# Autodesk Inventor assembly: Right Angle Structure
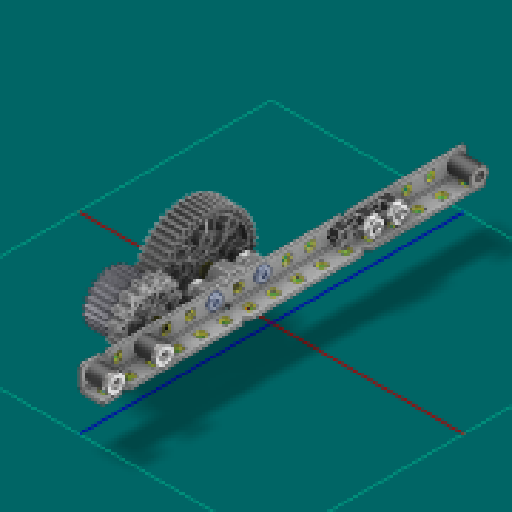
[picture p0: Inventor's stored thumbnail of the model, 512x512]
Saved by Autodesk Inventor 2025 (Build 290162000, 162)
## iProperties
Created: 2024-10-20
Part Number: Right Angle Structure
Document SubType Name: Assembly
Designer: Averey Ku
Author: Averey Ku
## Documents named in this file (18)
- C:\Users\avere\VEX\High Stakes\CAD\V2\Intake\Right Angle Structure\Right Angle Structure.iam
- C:\Users\avere\VEX\High Stakes\CAD\V2\Intake\Right Angle Structure\Right Alu Angle 1x1x16.ipt
- C:\Users\avere\VEX\High Stakes\CAD\V2\Intake\Right Angle Structure\Right Bearing Flat NScrew Slotted Offset.iam
- C:\Users\avere\VEX\High Stakes\CAD\ROBOPROS-CAD-Inventor\Motion\Spacers\Spacer Nylon .375 OD\NSpacer .375 OD x .500.ipt
- D:\VEX\High Stakes\CAD\ROBOPROS-CAD-Inventor\Motion\Spacers\Spacer Nylon .375 OD.ipt
- C:\Users\avere\VEX\High Stakes\CAD\ROBOPROS-CAD-Inventor\Motion\Spacers\Washer Steel\SWasher .375 OD x .015625.ipt
- D:\VEX\High Stakes\CAD\ROBOPROS-CAD-Inventor\Motion\Spacers\Washer Steel.ipt
- C:\Users\avere\VEX\High Stakes\CAD\V2\Intake\Right Angle Structure\Right HS Bearing Flat.ipt
- C:\Users\avere\VEX\High Stakes\CAD\ROBOPROS-CAD-Inventor\Structure\Hardware\Screw Shoulder Robosource\SScrew Shoulder Smooth .500 x .04.ipt
- D:\VEX\High Stakes\CAD\ROBOPROS-CAD-Inventor\Structure\Hardware\Screw Shoulder Robosource.ipt
- C:\Users\avere\VEX\High Stakes\CAD\ROBOPROS-CAD-Inventor\Structure\Hardware\Nut Nylon\Nut Nylon - White.ipt
- D:\VEX\High Stakes\CAD\ROBOPROS-CAD-Inventor\Structure\Hardware\Nut Nylon.ipt
- C:\Users\avere\VEX\High Stakes\CAD\ROBOPROS-CAD-Inventor\Motion\Spacers\Spacer Nylon .375 OD\NSpacer .375 OD x .375.ipt
- C:\Users\avere\VEX\High Stakes\CAD\ROBOPROS-CAD-Inventor\Motion\Spacers\Washer Steel\SWasher .375 OD x .062500.ipt
- C:\Users\avere\VEX\High Stakes\CAD\ROBOPROS-CAD-Inventor\Motion\Spacers\Washer Teflon\TWasher .375 OD x .04000.ipt
- D:\VEX\High Stakes\CAD\ROBOPROS-CAD-Inventor\Motion\Spacers\Washer Teflon.ipt
- C:\Users\avere\VEX\High Stakes\CAD\V2\Intake\Gearbox.iam
- Gearbox Left.iam
## Components (16 placed, 11 different names)
1. Right Alu Angle 1x1x16:1 — Mate:2, Mate:1, Flush:1, Mate:3, Insert:1, Insert:3, Mate:4, Insert:4, Insert:7, Insert:8, Insert:11, Insert:14, Insert:15
2. Right Bearing Flat NScrew Slotted Offset:1 [sub-assembly] — Mate:3, Insert:1
3. NSpacer .375 OD x .500:1 — Insert:3, Insert:2
4. SWasher .375 OD x .015625:1 — Insert:2
5. Right HS Bearing Flat:1 — Mate:4, Insert:4, Insert:5, Insert:6, Mate:6
6. SScrew Shoulder Smooth .500 x .04:1 — Insert:7
7. SScrew Shoulder Smooth .500 x .04:2 — Insert:8
8. Nut Nylon - White:1 — Insert:5
9. Nut Nylon - White:2 — Insert:6
10. NSpacer .375 OD x .375:2 — Insert:11, Insert:10
11. SWasher .375 OD x .062500:2 — Insert:10, Insert:9
12. TWasher .375 OD x .04000:1 — Insert:9
13. NSpacer .375 OD x .375:3 — Insert:14, Insert:13
14. SWasher .375 OD x .062500:3 — Insert:13, Insert:12
15. TWasher .375 OD x .04000:2 — Insert:12
16. Gearbox Left:1 [sub-assembly] — Insert:15, Mate:6
## Relationships (21: Insert 15, Mate 6)
- Mate:2: Right Alu Angle 1x1x16:1
- Mate:1: Right Alu Angle 1x1x16:1
- Flush:1 [Mate] (-101.6 mm): Right Alu Angle 1x1x16:1
- Mate:3: Right Alu Angle 1x1x16:1 ↔ Right Bearing Flat NScrew Slotted Offset:1
- Insert:1: Right Alu Angle 1x1x16:1 ↔ Right Bearing Flat NScrew Slotted Offset:1
- Insert:3: Right Alu Angle 1x1x16:1 ↔ NSpacer .375 OD x .500:1
- Insert:2: NSpacer .375 OD x .500:1 ↔ SWasher .375 OD x .015625:1
- Mate:4: Right Alu Angle 1x1x16:1 ↔ Right HS Bearing Flat:1
- Insert:4: Right Alu Angle 1x1x16:1 ↔ Right HS Bearing Flat:1
- Insert:7: Right Alu Angle 1x1x16:1 ↔ SScrew Shoulder Smooth .500 x .04:1
- Insert:8: Right Alu Angle 1x1x16:1 ↔ SScrew Shoulder Smooth .500 x .04:2
- Insert:5: Right HS Bearing Flat:1 ↔ Nut Nylon - White:1
- Insert:6: Right HS Bearing Flat:1 ↔ Nut Nylon - White:2
- Insert:11: Right Alu Angle 1x1x16:1 ↔ NSpacer .375 OD x .375:2
- Insert:10: NSpacer .375 OD x .375:2 ↔ SWasher .375 OD x .062500:2
- Insert:9: SWasher .375 OD x .062500:2 ↔ TWasher .375 OD x .04000:1
- Insert:14: Right Alu Angle 1x1x16:1 ↔ NSpacer .375 OD x .375:3
- Insert:13: NSpacer .375 OD x .375:3 ↔ SWasher .375 OD x .062500:3
- Insert:12: SWasher .375 OD x .062500:3 ↔ TWasher .375 OD x .04000:2
- Insert:15 (3.175 mm): Right Alu Angle 1x1x16:1 ↔ Gearbox Left:1
- Mate:6: Right HS Bearing Flat:1 ↔ Gearbox Left:1
